# Autodesk Inventor assembly: MouldAsm
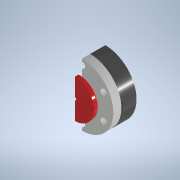
[picture p0: Inventor's stored thumbnail of the model, 180x180]
Saved by Autodesk Inventor 2020 (Build 240168000, 168)
## iProperties
Created: 2020-05-07
Part Number: MouldAsm
Document SubType Name: Assembly
Designer: Theo Cominotto
Author: Theo Cominotto
## Documents named in this file (4)
- C:\Users\Theo Cominotto\Dropbox\Beademingstoestel VUB\Beademingstoestel VUB-PEEP VALVE\Peep Custom\Silicone seal mould\MouldAsm.iam
- C:\Users\Theo Cominotto\Dropbox\Beademingstoestel VUB\Beademingstoestel VUB-PEEP VALVE\Peep Custom\Silicone seal mould\MouldBase.ipt
- C:\Users\Theo Cominotto\Dropbox\Beademingstoestel VUB\Beademingstoestel VUB-PEEP VALVE\Peep Custom\Silicone seal mould\MouldTop.ipt
- C:\Users\Theo Cominotto\Dropbox\Beademingstoestel VUB\Beademingstoestel VUB-PEEP VALVE\Peep Custom\Seal_M_TPU.ipt
## Components (3 placed, 3 different names)
1. MouldBase:1 — Mate:1, Mate:2, Mate:5
2. MouldTop:1 — Mate:1, Mate:2, Mate:3, Mate:4, Mate:5
3. Seal_M_TPU:1 — Mate:3
## Relationships (5: Mate 5)
- Mate:1: MouldBase:1 ↔ MouldTop:1
- Mate:2: MouldBase:1 ↔ MouldTop:1
- Mate:3: MouldTop:1 ↔ Seal_M_TPU:1
- Mate:4: MouldTop:1
- Mate:5: MouldBase:1 ↔ MouldTop:1
